# Autodesk Inventor assembly: SPARC-BOT
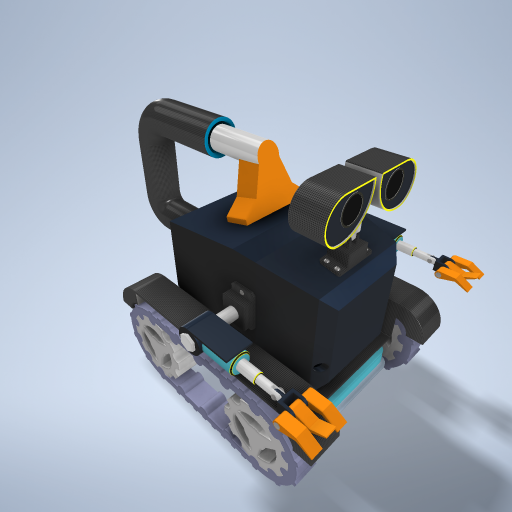
[picture p0: Inventor's stored thumbnail of the model, 512x512]
Saved by Autodesk Inventor 2024 (Build 280153000, 153)
## iProperties
Created: 2023-06-09
Part Number: SPARC-BOT
Document SubType Name: Assembly
Designer: vilas
Author: vilas
## Documents named in this file (23)
- D:\Parth Folder\ES101\Project\SPARC-BOT.iam
- D:\Parth Folder\ES101\Project\Scorpion Body - Internal.ipt
- D:\Parth Folder\ES101\Project\Pump.ipt
- D:\Parth Folder\ES101\Project\Pump_MIR.ipt
- D:\Parth Folder\ES101\Project\Hydraulic Arm.ipt
- D:\Parth Folder\ES101\Project\Claw Palm.ipt
- D:\Parth Folder\ES101\Project\Claw.ipt
- D:\Parth Folder\ES101\Project\Axis(2).ipt
- D:\Parth Folder\ES101\Project\Axis(1).ipt
- D:\Parth Folder\ES101\Project\Neck Base.ipt
- D:\Parth Folder\ES101\Project\Neck.ipt
- D:\Parth Folder\ES101\Project\Axis(3).ipt
- D:\Parth Folder\ES101\Project\body base.ipt
- D:\Parth Folder\ES101\Project\Cleaning Mop.ipt
- D:\Parth Folder\ES101\Project\Arduino.ipt
- D:\Parth Folder\ES101\Project\Head.ipt
- D:\Parth Folder\ES101\Project\UpperArm.ipt
- D:\Parth Folder\ES101\Project\vacuum.ipt
- D:\Parth Folder\ES101\Project\Battery.ipt
- D:\Parth Folder\ES101\Project\Wheels_Belt.iam
- D:\Parth Folder\ES101\Project\Vaccum pump.ipt
- D:\Parth Folder\ES101\Project\Vacuum noozle.ipt
- D:\Parth Folder\ES101\Project\Motor.ipt
## Components (54 placed, 22 different names)
1. Scorpion Body - Internal:1 — Mate:1, Mate:2, Mate:3, Mate:4, Mate:5, Mate:6, Mate:47, Mate:48, Mate:49, Mate:64, Mate:65, Mate:66, Mate:73, Flush:1, Mate:74, Mate:85, Mate:86, Mate:87, Mate:88, Mate:89, Mate:90, Mate:103, Flush:2, Mate:104, Mate:105, Flush:3
2. Pump:1 — Mate:1, Mate:2, Mate:3, Mate:27, Mate:28, Mate:29, Mate:30, Mate:31, Mate:32, Mate:33, Mate:34
3. Pump_MIR:1 — Mate:4, Mate:5, Mate:6, Mate:35, Mate:36, Mate:37, Mate:38, Mate:39, Mate:40, Mate:41, Mate:42
4. Hydraulic Arm:1 — Mate:7, Mate:8, Mate:25, Mate:99, Mate:100
5. Hydraulic Arm:2 — Mate:15, Mate:16, Mate:23, Mate:101, Mate:102
6. Claw Palm:1 — Mate:7, Mate:8, Mate:9, Mate:10, Mate:11, Mate:12, Mate:13, Mate:14, Mate:26
7. Claw Palm:2 — Mate:15, Mate:16, Mate:17, Mate:18, Mate:19, Mate:20, Mate:21, Mate:22, Mate:24
8. Claw:1 — Mate:17, Mate:18, Mate:43, Mate:44
9. Claw:2 — Mate:21, Mate:22
10. Claw:3 — Mate:19, Mate:20
11. Claw:4 — Mate:9, Mate:10
12. Claw:5 — Mate:13, Mate:14
13. Claw:6 — Mate:11, Mate:12, Mate:45, Mate:46
14. Axis(2):1 — Mate:23, Mate:24
15. Axis(2):2 — Mate:25, Mate:26
16. Axis(2):3 — Mate:30, Mate:34
17. Axis(2):4 — Mate:28, Mate:33
18. Axis(2):5 — Mate:27, Mate:31
19. Axis(2):6 — Mate:29, Mate:32
20. Axis(2):7 — Mate:36, Mate:41
21. Axis(2):8 — Mate:37, Mate:39
22. Axis(2):9 — Mate:35, Mate:42
23. Axis(2):10 — Mate:38, Mate:40
24. Axis(1):1 — Mate:45, Mate:46
25. Axis(1):2 — Mate:43, Mate:44
26. Neck Base:1 — Mate:47, Mate:48, Mate:49, Mate:50, Mate:51, Mate:52, Mate:53, Mate:54, Mate:55, Mate:56, Mate:57, Mate:59, Mate:61, Mate:62, Mate:63
27. Axis(2):11 — Mate:50, Mate:56
28. Axis(2):12 — Mate:53, Mate:55
29. Axis(2):13 — Mate:52, Mate:54
30. Axis(2):14 — Mate:51, Mate:57
31. Neck:1 — Mate:59, Mate:62, Mate:75, Mate:76
32. Axis(3):1 — Mate:61, Mate:63
33. body base:1 — Mate:64, Mate:65, Mate:66, Mate:67, Mate:68, Mate:69, Mate:70, Mate:71, Mate:72
34. Cleaning Mop:1 — Mate:71, Mate:72, Mate:106, Mate:107, Mate:108, Mate:109, Mate:110, Mate:111, Mate:116, Mate:117, Mate:118, Mate:119, Mate:120, Mate:121, Mate:122, Mate:123
35. Axis(2):15 — Mate:67, Mate:69
36. Axis(2):16 — Mate:68, Mate:70
37. Arduino:1 — Mate:73, Flush:1, Mate:74
38. Head:1 — Mate:75, Mate:76
39. UpperArm:1 — Mate:85, Mate:86, Mate:87, Mate:91, Mate:92, Mate:93, Mate:94, Mate:99, Mate:100
40. UpperArm:2 — Mate:88, Mate:89, Mate:90, Mate:95, Mate:96, Mate:97, Mate:98, Mate:101, Mate:102
41. Axis(2):17 — Mate:91, Mate:92
42. Axis(2):18 — Mate:93, Mate:94
43. Axis(2):19 — Mate:95, Mate:96
44. Axis(2):20 — Mate:97, Mate:98
45. vacuum:1 — Mate:103, Flush:2, Mate:112, Mate:113, Mate:114, Mate:115
46. Battery:1 — Mate:104, Mate:105, Flush:3
47. Wheels_Belt:1 [sub-assembly] — Mate:109, Mate:110, Mate:111
48. Wheels_Belt:2 [sub-assembly] — Mate:106, Mate:107, Mate:108
49. Vaccum pump:1 — Mate:112, Mate:113
50. Vacuum noozle:1 — Mate:114, Mate:115
51. Motor:1 — Mate:122, Mate:123
52. Motor:2 — Mate:120, Mate:121
53. Motor:3 — Mate:116, Mate:117
54. Motor:4 — Mate:118, Mate:119
## Relationships (116: Mate 113, Flush 3)
- Mate:1: Scorpion Body - Internal:1 ↔ Pump:1
- Mate:2: Scorpion Body - Internal:1 ↔ Pump:1
- Mate:3: Scorpion Body - Internal:1 ↔ Pump:1
- Mate:4: Scorpion Body - Internal:1 ↔ Pump_MIR:1
- Mate:5: Scorpion Body - Internal:1 ↔ Pump_MIR:1
- Mate:6: Scorpion Body - Internal:1 ↔ Pump_MIR:1
- Mate:7: Hydraulic Arm:1 ↔ Claw Palm:1
- Mate:8: Hydraulic Arm:1 ↔ Claw Palm:1
- Mate:9: Claw Palm:1 ↔ Claw:4
- Mate:10: Claw Palm:1 ↔ Claw:4
- Mate:11: Claw Palm:1 ↔ Claw:6
- Mate:12: Claw Palm:1 ↔ Claw:6
- Mate:13: Claw Palm:1 ↔ Claw:5
- Mate:14: Claw Palm:1 ↔ Claw:5
- Mate:15: Hydraulic Arm:2 ↔ Claw Palm:2
- Mate:16: Hydraulic Arm:2 ↔ Claw Palm:2
- Mate:17: Claw Palm:2 ↔ Claw:1
- Mate:18: Claw Palm:2 ↔ Claw:1
- Mate:19: Claw Palm:2 ↔ Claw:3
- Mate:20: Claw Palm:2 ↔ Claw:3
- Mate:21: Claw Palm:2 ↔ Claw:2
- Mate:22: Claw Palm:2 ↔ Claw:2
- Mate:23: Hydraulic Arm:2 ↔ Axis(2):1
- Mate:24 (5 mm): Claw Palm:2 ↔ Axis(2):1
- Mate:25: Hydraulic Arm:1 ↔ Axis(2):2
- Mate:26 (5 mm): Claw Palm:1 ↔ Axis(2):2
- Mate:27: Pump:1 ↔ Axis(2):5
- Mate:28: Pump:1 ↔ Axis(2):4
- Mate:29: Pump:1 ↔ Axis(2):6
- Mate:30: Pump:1 ↔ Axis(2):3
- Mate:31: Pump:1 ↔ Axis(2):5
- Mate:32: Pump:1 ↔ Axis(2):6
- Mate:33: Pump:1 ↔ Axis(2):4
- Mate:34: Pump:1 ↔ Axis(2):3
- Mate:35: Pump_MIR:1 ↔ Axis(2):9
- Mate:36: Pump_MIR:1 ↔ Axis(2):7
- Mate:37: Pump_MIR:1 ↔ Axis(2):8
- Mate:38: Pump_MIR:1 ↔ Axis(2):10
- Mate:39: Pump_MIR:1 ↔ Axis(2):8
- Mate:40: Pump_MIR:1 ↔ Axis(2):10
- Mate:41: Pump_MIR:1 ↔ Axis(2):7
- Mate:42: Pump_MIR:1 ↔ Axis(2):9
- Mate:43: Claw:1 ↔ Axis(1):2
- Mate:44: Claw:1 ↔ Axis(1):2
- Mate:45: Claw:6 ↔ Axis(1):1
- Mate:46: Claw:6 ↔ Axis(1):1
- Mate:47: Scorpion Body - Internal:1 ↔ Neck Base:1
- Mate:48: Scorpion Body - Internal:1 ↔ Neck Base:1
- Mate:49: Scorpion Body - Internal:1 ↔ Neck Base:1
- Mate:50: Neck Base:1 ↔ Axis(2):11
- Mate:51: Neck Base:1 ↔ Axis(2):14
- Mate:52: Neck Base:1 ↔ Axis(2):13
- Mate:53: Neck Base:1 ↔ Axis(2):12
- Mate:54: Neck Base:1 ↔ Axis(2):13
- Mate:55: Neck Base:1 ↔ Axis(2):12
- Mate:56: Neck Base:1 ↔ Axis(2):11
- Mate:57: Neck Base:1 ↔ Axis(2):14
- Mate:59: Neck Base:1 ↔ Neck:1
- Mate:61: Neck Base:1 ↔ Axis(3):1
- Mate:62: Neck Base:1 ↔ Neck:1
- Mate:63: Neck Base:1 ↔ Axis(3):1
- Mate:64: Scorpion Body - Internal:1 ↔ body base:1
- Mate:65: Scorpion Body - Internal:1 ↔ body base:1
- Mate:66: Scorpion Body - Internal:1 ↔ body base:1
- Mate:67: body base:1 ↔ Axis(2):15
- Mate:68: body base:1 ↔ Axis(2):16
- Mate:69: body base:1 ↔ Axis(2):15
- Mate:70: body base:1 ↔ Axis(2):16
- Mate:71: body base:1 ↔ Cleaning Mop:1
- Mate:72: body base:1 ↔ Cleaning Mop:1
- Mate:73: Scorpion Body - Internal:1 ↔ Arduino:1
- Flush:1: Scorpion Body - Internal:1 ↔ Arduino:1
- Mate:74 (30 mm): Scorpion Body - Internal:1 ↔ Arduino:1
- Mate:75: Neck:1 ↔ Head:1
- Mate:76: Neck:1 ↔ Head:1
- Mate:85: Scorpion Body - Internal:1 ↔ UpperArm:1
- Mate:86: Scorpion Body - Internal:1 ↔ UpperArm:1
- Mate:87: Scorpion Body - Internal:1 ↔ UpperArm:1
- Mate:88: Scorpion Body - Internal:1 ↔ UpperArm:2
- Mate:89: Scorpion Body - Internal:1 ↔ UpperArm:2
- Mate:90: Scorpion Body - Internal:1 ↔ UpperArm:2
- Mate:91: UpperArm:1 ↔ Axis(2):17
- Mate:92: UpperArm:1 ↔ Axis(2):17
- Mate:93: UpperArm:1 ↔ Axis(2):18
- Mate:94: UpperArm:1 ↔ Axis(2):18
- Mate:95: UpperArm:2 ↔ Axis(2):19
- Mate:96: UpperArm:2 ↔ Axis(2):19
- Mate:97: UpperArm:2 ↔ Axis(2):20
- Mate:98: UpperArm:2 ↔ Axis(2):20
- Mate:99: Hydraulic Arm:1 ↔ UpperArm:1
- Mate:100: Hydraulic Arm:1 ↔ UpperArm:1
- Mate:101: Hydraulic Arm:2 ↔ UpperArm:2
- Mate:102: Hydraulic Arm:2 ↔ UpperArm:2
- Mate:103: Scorpion Body - Internal:1 ↔ vacuum:1
- Flush:2: Scorpion Body - Internal:1 ↔ vacuum:1
- Mate:104: Scorpion Body - Internal:1 ↔ Battery:1
- Mate:105 (30 mm): Scorpion Body - Internal:1 ↔ Battery:1
- Flush:3: Scorpion Body - Internal:1 ↔ Battery:1
- Mate:106: Cleaning Mop:1 ↔ Wheels_Belt:2
- Mate:107: Cleaning Mop:1 ↔ Wheels_Belt:2
- Mate:108: Cleaning Mop:1 ↔ Wheels_Belt:2
- Mate:109: Cleaning Mop:1 ↔ Wheels_Belt:1
- Mate:110: Cleaning Mop:1 ↔ Wheels_Belt:1
- Mate:111: Cleaning Mop:1 ↔ Wheels_Belt:1
- Mate:112: vacuum:1 ↔ Vaccum pump:1
- Mate:113: vacuum:1 ↔ Vaccum pump:1
- Mate:114: vacuum:1 ↔ Vacuum noozle:1
- Mate:115: vacuum:1 ↔ Vacuum noozle:1
- Mate:116: Cleaning Mop:1 ↔ Motor:3
- Mate:117: Cleaning Mop:1 ↔ Motor:3
- Mate:118: Cleaning Mop:1 ↔ Motor:4
- Mate:119: Cleaning Mop:1 ↔ Motor:4
- Mate:120: Cleaning Mop:1 ↔ Motor:2
- Mate:121: Cleaning Mop:1 ↔ Motor:2
- Mate:122: Cleaning Mop:1 ↔ Motor:1
- Mate:123: Cleaning Mop:1 ↔ Motor:1
